# Autodesk Inventor assembly: platform_0606_fig2_ratio10
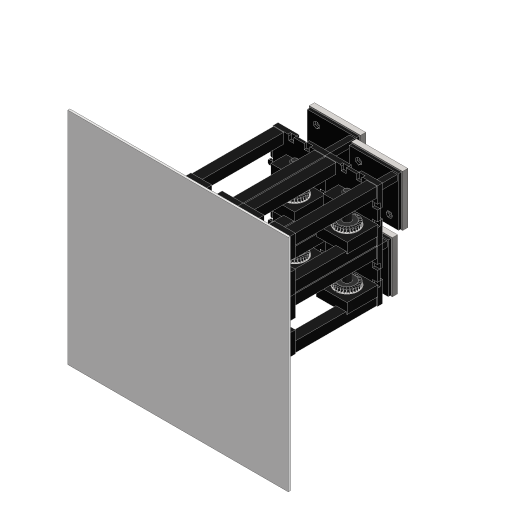
[picture p0: Inventor's stored thumbnail of the model, 512x512]
Saved by Autodesk Inventor 2024 (Build 280153000, 153)
## iProperties
Created: 2024-06-06
Part Number: platform_0606_fig2_ratio10
Document SubType Name: Assembly
Designer: admin
Author: admin
## Documents named in this file (14)
- C:\Users\admin\OneDrive\文件\碩士研究\prototype\plane_unit_0606\platform_0606_fig2_ladder.iam
- C:\Users\admin\OneDrive\文件\碩士研究\prototype\plane_unit_0606\one_way_bearing.ipt
- C:\Users\admin\OneDrive\文件\碩士研究\prototype\plane_unit_0606\printer_base_plane.ipt
- C:\Users\admin\OneDrive\文件\碩士研究\prototype\plane_unit_0606\rod_1221.ipt
- C:\Users\admin\OneDrive\文件\碩士研究\prototype\plane_unit_0606\iron_plate.ipt
- C:\Users\admin\OneDrive\文件\碩士研究\prototype\plane_unit_0606\plane_unit_1121.ipt
- C:\Users\admin\OneDrive\文件\碩士研究\prototype\plane_unit_0606\gear_pin_1222_.ipt
- C:\Users\admin\OneDrive\文件\碩士研究\prototype\plane_unit_0606\Template_ladder_2.ipt
- C:\Users\admin\OneDrive\文件\碩士研究\prototype\plane_unit_0606\iron_plate_CPY.ipt
- C:\Users\admin\OneDrive\文件\碩士研究\prototype\plane_unit_0606\rod_1221_CPY.ipt
- C:\Users\admin\OneDrive\文件\碩士研究\prototype\plane_unit_0606\iron_plate_CPY1.ipt
- C:\Users\admin\OneDrive\文件\碩士研究\prototype\plane_unit_0606\rod_1221_CPY1.ipt
- C:\Users\admin\OneDrive\文件\碩士研究\prototype\plane_unit_0606\iron_plate_CPY2.ipt
- C:\Users\admin\OneDrive\文件\碩士研究\prototype\plane_unit_0606\rod_1221_CPY2.ipt
## Components (22 placed, 13 different names)
1. printer_base_plane:1 — 貼合:1, 齊平:1, 齊平:2, 齊平:7, 齊平:8, 齊平:9, 齊平:10, 齊平:11, 齊平:23, 齊平:24
2. rod_1221:1 — 貼合:7, 貼合:8, 貼合:9, 貼合:10, 貼合:11
3. iron_plate:1 — 貼合:9, 貼合:10, 貼合:11, 齊平:5, 貼合:22
4. Template_ladder_2:1 — 齊平:5, 齊平:25, 貼合:21, 貼合:22, 貼合:23, 貼合:24
5. iron_plate_CPY:1 — 貼合:12, 貼合:13, 貼合:14, 貼合:23
6. rod_1221_CPY:1 — 貼合:12, 貼合:13, 貼合:14, 齊平:10, 齊平:11
7. iron_plate_CPY1:1 — 貼合:15, 貼合:16, 貼合:17, 貼合:24
8. rod_1221_CPY1:1 — 貼合:15, 貼合:16, 貼合:17, 齊平:9, 齊平:23
9. iron_plate_CPY2:1 — 貼合:18, 貼合:19, 貼合:20, 齊平:24, 齊平:25, 貼合:21
10. rod_1221_CPY2:1 — 貼合:18, 貼合:19, 貼合:20, 齊平:7, 齊平:8
11. one_way_bearing:1 — 貼合:2, 齊平:3, 貼合:3, 貼合:4
12. plane_unit_1121:1 — 貼合:1, 齊平:1, 齊平:2, 貼合:2, 齊平:3, 貼合:7, 貼合:8
13. gear_pin_1222_:1 — 貼合:3, 貼合:4
14. one_way_bearing:2
15. plane_unit_1121:2
16. gear_pin_1222_:2
17. one_way_bearing:3
18. plane_unit_1121:3
19. gear_pin_1222_:3
20. one_way_bearing:4
21. plane_unit_1121:4
22. gear_pin_1222_:4
## Component patterns: (4 elements, first: one_way_bearing:1 + plane_unit_1121:1 + gear_pin_1222_:1)
## Relationships (34: Mate 22, Flush 12)
- 貼合:1 [Mate]: printer_base_plane:1 ↔ plane_unit_1121:1
- 齊平:1 [Flush] (5 mm): printer_base_plane:1 ↔ plane_unit_1121:1
- 齊平:2 [Flush] (5 mm): printer_base_plane:1 ↔ plane_unit_1121:1
- 貼合:2 [Mate]: one_way_bearing:1 ↔ plane_unit_1121:1
- 齊平:3 [Flush]: one_way_bearing:1 ↔ plane_unit_1121:1
- 貼合:3 [Mate]: one_way_bearing:1 ↔ gear_pin_1222_:1
- 貼合:4 [Mate]: one_way_bearing:1 ↔ gear_pin_1222_:1
- 貼合:7 [Mate] (0.2 mm): rod_1221:1 ↔ plane_unit_1121:1
- 貼合:8 [Mate] (0.2 mm): rod_1221:1 ↔ plane_unit_1121:1
- 貼合:9 [Mate]: rod_1221:1 ↔ iron_plate:1
- 貼合:10 [Mate]: rod_1221:1 ↔ iron_plate:1
- 貼合:11 [Mate]: rod_1221:1 ↔ iron_plate:1
- 貼合:12 [Mate]: iron_plate_CPY:1 ↔ rod_1221_CPY:1
- 貼合:13 [Mate]: iron_plate_CPY:1 ↔ rod_1221_CPY:1
- 貼合:14 [Mate]: iron_plate_CPY:1 ↔ rod_1221_CPY:1
- 貼合:15 [Mate]: iron_plate_CPY1:1 ↔ rod_1221_CPY1:1
- 貼合:16 [Mate]: iron_plate_CPY1:1 ↔ rod_1221_CPY1:1
- 貼合:17 [Mate]: iron_plate_CPY1:1 ↔ rod_1221_CPY1:1
- 貼合:18 [Mate]: iron_plate_CPY2:1 ↔ rod_1221_CPY2:1
- 貼合:19 [Mate]: iron_plate_CPY2:1 ↔ rod_1221_CPY2:1
- 貼合:20 [Mate]: iron_plate_CPY2:1 ↔ rod_1221_CPY2:1
- 齊平:5 [Flush] (4 mm): iron_plate:1 ↔ Template_ladder_2:1
- 齊平:7 [Flush] (7.7 mm): printer_base_plane:1 ↔ rod_1221_CPY2:1
- 齊平:8 [Flush] (58.7 mm): printer_base_plane:1 ↔ rod_1221_CPY2:1
- 齊平:9 [Flush] (58.7 mm): printer_base_plane:1 ↔ rod_1221_CPY1:1
- 齊平:10 [Flush] (7.7 mm): printer_base_plane:1 ↔ rod_1221_CPY:1
- 齊平:11 [Flush] (58.7 mm): printer_base_plane:1 ↔ rod_1221_CPY:1
- 齊平:23 [Flush] (58.7 mm): printer_base_plane:1 ↔ rod_1221_CPY1:1
- 齊平:24 [Flush] (-110 mm): printer_base_plane:1 ↔ iron_plate_CPY2:1
- 齊平:25 [Flush] (1 mm): Template_ladder_2:1 ↔ iron_plate_CPY2:1
- 貼合:21 [Mate]: Template_ladder_2:1 ↔ iron_plate_CPY2:1
- 貼合:22 [Mate]: iron_plate:1 ↔ Template_ladder_2:1
- 貼合:23 [Mate]: Template_ladder_2:1 ↔ iron_plate_CPY:1
- 貼合:24 [Mate]: Template_ladder_2:1 ↔ iron_plate_CPY1:1
